# Autodesk Inventor assembly: SDS MK4i Swerve Module NEOS_2.0
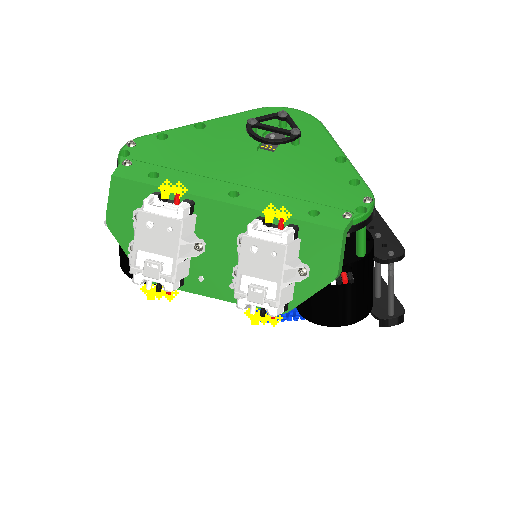
[picture p0: Inventor's stored thumbnail of the model, 512x512]
Saved by Autodesk Inventor 2023 (Build 270158000, 158)
## iProperties
Created: 2023-03-28
Part Number: SDS MK4i Swerve Module NEOS_2.0
Document SubType Name: Assembly
Designer: jackc
Mass: 1358.74 g
Surface Area: 6264.05 cm^2
Volume: 1128.55 cm^3
Density: 1.20396 g/cm^3
Author: jackc
## Documents named in this file (10)
- J:\My Drive\1939\2_Design\2023-2024\Parts\Swerve\SDS MK4i Swerve Module NEOS_2.0.iam
- J:\My Drive\1939\2_Design\2023-2024\Parts\Swerve\NEO Drive Gear.iam
- J:\My Drive\1939\2_Design\2023-2024\Parts\Swerve\NEO Turn Gear.iam
- J:\My Drive\1939\2_Design\2023-2024\Parts\Swerve\SDS MK4i Swerve Module, unpopulated.iam
- J:\My Drive\1939\2_Design\2023-2024\Parts\Motors\NEO Motor.ipt
- J:\My Drive\1939\2_Design\2023-2024\Parts\Electronics\Motor Controllers\REV-11-2158-Spark-MAX.ipt
- J:\My Drive\1939\2_Design\2023-2024\Parts\Electronics\Motor Controllers\REV-21-2151_SPM_Mount.ipt
- J:\My Drive\1939\2_Design\2023-2024\Parts\Printed Parts\Module_SPM_Mount_2.0_SMM.ipt
- J:\My Drive\1939\2_Design\2023-2024\Parts\Hardware\#8\Screw 8-32 x 0.750_.ipt
- J:\My Drive\1939\2_Design\2023-2024\Parts\Printed Parts\Module_SPM_Mount_2.1_Top.ipt
## Components (21 placed, 9 different names)
1. NEO Drive Gear:1 [sub-assembly]
2. NEO Turn Gear:1 [sub-assembly]
3. SDS MK4i Swerve Module, unpopulated:1 [sub-assembly] — Mate:13, Mate:14, Mate:16, Mate:17, Mate:18, Mate:19, Mate:31, Mate:32, Mate:46
4. NEO Motor:1 — Mate:13, Mate:14, Mate:19
5. NEO Motor:2 — Mate:16, Mate:17, Mate:18
6. Module_SPM_Mount_2.1_Top:1
7. REV-11-2158-Spark-MAX:3 — Mate:22, Flush:2, Mate:24, Mate:29, Mate:30
8. REV-11-2158-Spark-MAX:2 — Mate:23, Flush:1, Flush:2, Flush:3, Mate:24, Mate:26, Mate:27
9. REV-21-2151_SPM_Mount:1 — Mate:28, Mate:29, Mate:30, Mate:37, Mate:38, Mate:39, Mate:40, Mate:43
10. REV-21-2151_SPM_Mount:2 — Mate:25, Mate:26, Mate:27, Mate:41, Mate:42, Mate:44
11. Module_SPM_Mount_2.0_SMM:1 — Mate:22, Mate:23, Flush:1, Flush:3, Mate:25, Mate:28, Mate:31, Mate:32, Mate:33, Mate:34, Mate:35, Mate:36
12. Screw 8-32 x 0.750_:1 — Mate:33, Mate:34
13. Screw 8-32 x 0.750_:2 — Mate:35, Mate:36
14. Screw 8-32 x 0.750_:3 — Mate:37, Mate:38
15. Screw 8-32 x 0.750_:4 — Flush:4, Mate:39, Mate:40
16. Screw 8-32 x 0.750_:5 — Flush:4, Flush:5, Mate:41
17. Screw 8-32 x 0.750_:6 — Flush:5, Flush:6, Mate:44
18. Screw 8-32 x 0.750_:7 — Flush:6, Flush:7, Mate:43
19. Screw 8-32 x 0.750_:8 — Flush:7, Mate:42
20. Screw 8-32 x 0.750_:9 — Mate:46
21. Screw 8-32 x 0.750_:10
## Relationships (45: Mate 36, Flush 7, Angle 2)
- [Mate]: SDS MK4i Swerve Module, unpopulated:1 ↔ Module_SPM_Mount_2.1_Top:1
- [Mate]: SDS MK4i Swerve Module, unpopulated:1 ↔ Module_SPM_Mount_2.1_Top:1
- [Angle] (180 deg): SDS MK4i Swerve Module, unpopulated:1 ↔ Module_SPM_Mount_2.1_Top:1
- [Mate]: SDS MK4i Swerve Module, unpopulated:1 ↔ Module_SPM_Mount_2.1_Top:1
- Mate:13: SDS MK4i Swerve Module, unpopulated:1 ↔ NEO Motor:1
- Mate:14: SDS MK4i Swerve Module, unpopulated:1 ↔ NEO Motor:1
- Mate:16: SDS MK4i Swerve Module, unpopulated:1 ↔ NEO Motor:2
- Mate:17: SDS MK4i Swerve Module, unpopulated:1 ↔ NEO Motor:2
- Mate:18: SDS MK4i Swerve Module, unpopulated:1 ↔ NEO Motor:2
- Mate:19: SDS MK4i Swerve Module, unpopulated:1 ↔ NEO Motor:1
- Mate:22: REV-11-2158-Spark-MAX:3 ↔ Module_SPM_Mount_2.0_SMM:1
- Mate:23: REV-11-2158-Spark-MAX:2 ↔ Module_SPM_Mount_2.0_SMM:1
- Flush:1 (3.175 mm): REV-11-2158-Spark-MAX:2 ↔ Module_SPM_Mount_2.0_SMM:1
- Flush:2: REV-11-2158-Spark-MAX:3 ↔ REV-11-2158-Spark-MAX:2
- Flush:3 (35.3441 mm): REV-11-2158-Spark-MAX:2 ↔ Module_SPM_Mount_2.0_SMM:1
- Mate:24 (50.8 mm): REV-11-2158-Spark-MAX:3 ↔ REV-11-2158-Spark-MAX:2
- Mate:25: REV-21-2151_SPM_Mount:2 ↔ Module_SPM_Mount_2.0_SMM:1
- Mate:26: REV-11-2158-Spark-MAX:2 ↔ REV-21-2151_SPM_Mount:2
- Mate:27: REV-11-2158-Spark-MAX:2 ↔ REV-21-2151_SPM_Mount:2
- Mate:28: REV-21-2151_SPM_Mount:1 ↔ Module_SPM_Mount_2.0_SMM:1
- Mate:29: REV-11-2158-Spark-MAX:3 ↔ REV-21-2151_SPM_Mount:1
- Mate:30: REV-11-2158-Spark-MAX:3 ↔ REV-21-2151_SPM_Mount:1
- Mate:31: SDS MK4i Swerve Module, unpopulated:1 ↔ Module_SPM_Mount_2.0_SMM:1
- Mate:32: SDS MK4i Swerve Module, unpopulated:1 ↔ Module_SPM_Mount_2.0_SMM:1
- [Angle] (180 deg): Module_SPM_Mount_2.1_Top:1 ↔ Module_SPM_Mount_2.0_SMM:1
- Mate:33: Module_SPM_Mount_2.0_SMM:1 ↔ Screw 8-32 x 0.750_:1
- Mate:34: Module_SPM_Mount_2.0_SMM:1 ↔ Screw 8-32 x 0.750_:1
- Mate:35: Module_SPM_Mount_2.0_SMM:1 ↔ Screw 8-32 x 0.750_:2
- Mate:36: Module_SPM_Mount_2.0_SMM:1 ↔ Screw 8-32 x 0.750_:2
- Mate:37: REV-21-2151_SPM_Mount:1 ↔ Screw 8-32 x 0.750_:3
- Mate:38: REV-21-2151_SPM_Mount:1 ↔ Screw 8-32 x 0.750_:3
- Flush:4: Screw 8-32 x 0.750_:4 ↔ Screw 8-32 x 0.750_:5
- Flush:5: Screw 8-32 x 0.750_:5 ↔ Screw 8-32 x 0.750_:6
- Flush:6: Screw 8-32 x 0.750_:6 ↔ Screw 8-32 x 0.750_:7
- Flush:7: Screw 8-32 x 0.750_:7 ↔ Screw 8-32 x 0.750_:8
- Mate:39: REV-21-2151_SPM_Mount:1 ↔ Screw 8-32 x 0.750_:4
- Mate:40: REV-21-2151_SPM_Mount:1 ↔ Screw 8-32 x 0.750_:4
- Mate:41: REV-21-2151_SPM_Mount:2 ↔ Screw 8-32 x 0.750_:5
- Mate:42: REV-21-2151_SPM_Mount:2 ↔ Screw 8-32 x 0.750_:8
- Mate:43: REV-21-2151_SPM_Mount:1 ↔ Screw 8-32 x 0.750_:7
- Mate:44: REV-21-2151_SPM_Mount:2 ↔ Screw 8-32 x 0.750_:6
- [Mate]: Module_SPM_Mount_2.1_Top:1 ↔ Screw 8-32 x 0.750_:9
- Mate:46: SDS MK4i Swerve Module, unpopulated:1 ↔ Screw 8-32 x 0.750_:9
- [Mate]: Module_SPM_Mount_2.1_Top:1 ↔ Screw 8-32 x 0.750_:10
- [Mate]: Module_SPM_Mount_2.1_Top:1 ↔ Screw 8-32 x 0.750_:10
